# Autodesk Inventor assembly: 50mm_EDF
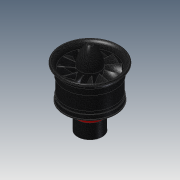
[picture p0: Inventor's stored thumbnail of the model, 180x180]
Saved by Autodesk Inventor 2015 (Build 190159000, 159)
## iProperties
Created: 2017-11-27
Part Number: 50mm_EDF
Document SubType Name: Assembly
Designer: USER
Author: USER
## Documents named in this file (5)
- C:\Users\USER\Desktop\Drone\50mm_EDF_3D\50mm_EDF.iam
- C:\Users\USER\Desktop\Drone\50mm_EDF_3D\motor.ipt
- C:\Users\USER\Desktop\Drone\50mm_EDF_3D\風扇本體.ipt
- C:\Users\USER\Desktop\Drone\50mm_EDF_3D\風扇頭.ipt
- C:\Users\USER\Desktop\Drone\50mm_EDF_3D\扇葉.ipt
## Components (4 placed, 4 different names)
1. motor:1 — 貼合:1, 貼合:2, 旋轉:1
2. 風扇本體:1 — 貼合:1, 貼合:2, 貼合:3, 貼合:4, 旋轉:2
3. 風扇頭:1 — 貼合:3, 貼合:4, 貼合:5, 貼合:6, 貼合:7, 旋轉:2
4. 扇葉:1 — 貼合:5, 貼合:6, 旋轉:1
## Relationships (9: Mate 7, RelateRotation 2)
- 貼合:1 [Mate]: motor:1 ↔ 風扇本體:1
- 貼合:2 [Mate]: motor:1 ↔ 風扇本體:1
- 貼合:3 [Mate]: 風扇本體:1 ↔ 風扇頭:1
- 貼合:4 [Mate] (-3.7 mm): 風扇本體:1 ↔ 風扇頭:1
- 貼合:5 [Mate]: 風扇頭:1 ↔ 扇葉:1
- 貼合:6 [Mate]: 風扇頭:1 ↔ 扇葉:1
- 貼合:7 [Mate]: 風扇頭:1
- 旋轉:1 [RelateRotation] (0.844 ul): motor:1 ↔ 扇葉:1
- 旋轉:2 [RelateRotation] (1 ul): 風扇本體:1 ↔ 風扇頭:1
